# Autodesk Inventor assembly: formed_machine
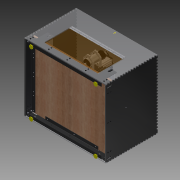
[picture p0: Inventor's stored thumbnail of the model, 180x180]
Saved by Autodesk Inventor 2014 (Build 180170000, 170)
## iProperties
Created: 2013-05-31
Part Number: formed_machine
Document SubType Name: Assembly
Designer: Edward
Mass: 12074.1 g
Surface Area: 21541.8 cm^2
Volume: 5793.23 cm^3
Density: 2.08417 g/cm^3
Author: Edward
## Documents named in this file (21)
- C:\Users\Edward\Desktop\Shapeoko_2.0_collection\Shapeoko_formed\Workgroups\Workgroup\shapeoko_v2_0.iam
- C:\Users\Edward\Desktop\Shapeoko_2.0_collection\Shapeoko_formed\Workgroups\Workgroup\formed_front_back.ipt
- C:\Users\Edward\Desktop\Shapeoko_2.0_collection\Shapeoko_formed\Workgroups\Workgroup\S2_MS500.ipt
- C:\Users\Edward\Desktop\Shapeoko_2.0_collection\Shapeoko_formed\Workgroups\Workgroup\plate_assembly_stacked.iam
- C:\Users\Edward\Desktop\Shapeoko_2.0_collection\Shapeoko_formed\Workgroups\Workgroup\formed_right_left.ipt
- C:\Users\Edward\Desktop\Shapeoko_2.0_collection\Shapeoko_formed\Workgroups\Workgroup\sectional_wasteboard.ipt
- C:\Users\Edward\Desktop\Shapeoko_2.0_collection\Shapeoko_formed\Workgroups\Workgroup\23015T82_leveling_feet.ipt
- C:\Users\Edward\Desktop\Shapeoko_2.0_collection\Shapeoko_formed\Workgroups\Workgroup\z-axis_assembly.iam
- C:\Users\Edward\Desktop\Shapeoko_2.0_collection\Shapeoko_formed\Workgroups\Workgroup\SM-H03.ipt
- C:\Users\Edward\Desktop\Shapeoko_2.0_collection\Shapeoko_formed\Workgroups\Workgroup\SM-H04.ipt
- C:\Users\Edward\Desktop\Shapeoko_2.0_collection\Shapeoko_formed\Workgroups\Workgroup\91239A228.ipt
- C:\Users\Edward\Desktop\Shapeoko_2.0_collection\Shapeoko_formed\Workgroups\Workgroup\belt_clip_assembly.iam
- C:\Users\Edward\Desktop\Shapeoko_2.0_collection\Shapeoko_formed\Workgroups\Workgroup\97349A200.ipt
- C:\Users\Edward\Desktop\Shapeoko_2.0_collection\Shapeoko_formed\Workgroups\Workgroup\GT2_XY_belting.ipt
- C:\Users\Edward\Desktop\Shapeoko_2.0_collection\Shapeoko_formed\Workgroups\Workgroup\fr.ipt
- C:\Users\Edward\Desktop\Shapeoko_2.0_collection\Shapeoko_formed\Workgroups\Workgroup\hblsd_assembly.iam
- C:\Users\Edward\Desktop\Shapeoko_2.0_collection\Shapeoko_formed\Workgroups\Workgroup\case_right.ipt
- C:\Users\Edward\Desktop\Shapeoko_2.0_collection\Shapeoko_formed\Workgroups\Workgroup\case_front.ipt
- C:\Users\Edward\Desktop\Shapeoko_2.0_collection\Shapeoko_formed\Workgroups\Workgroup\case_rear.ipt
- C:\Users\Edward\Desktop\Shapeoko_2.0_collection\Shapeoko_formed\Workgroups\Workgroup\Imported Components\1569A107\1569A107.ipt
- C:\Users\Edward\Desktop\Shapeoko_2.0_collection\Shapeoko_formed\Workgroups\Workgroup\case_door.ipt
## Components (159 placed, 20 different names)
1. formed_front_back:1 — Angle:1, Angle:2, Flush:4, Mate:16, Flush:5, Insert:9, Insert:10, Mate:22, Mate:23, Flush:10, Flush:11, Flush:12, Flush:13, Flush:14, Flush:15, Mate:31, Insert:55, Insert:56, Insert:57, Mate:38, Flush:22
2. S2_MS500:1 — Angle:2, Mate:1, Flush:1, Insert:6, Insert:17, Insert:18, Mate:23, Flush:10, Flush:13, Mate:24, Mate:28, Mate:30, Flush:16, Mate:43, Flush:26
3. plate_assembly_stacked:1 [sub-assembly] — Mate:1, Flush:1, Insert:4, Angle:3, Mate:36
4. S2_MS500:2 — Angle:1, Mate:2, Flush:2, Insert:5, Insert:23, Insert:24, Mate:22, Flush:11, Flush:12, Mate:25, Mate:27, Mate:41
5. plate_assembly_stacked:2 [sub-assembly] — Mate:2, Flush:2, Insert:3, Mate:34
6. S2_MS500:3 — Insert:3, Insert:4, Mate:20, Flush:7, Angle:3, Insert:37, Insert:38, Insert:40, Insert:42, Mate:21, Mate:26, Mate:29, Mate:33, Mate:35, Flush:18, Flush:19, Mate:42, Flush:25
7. formed_front_back:2 — Insert:5, Insert:6, Mate:14, Mate:15, Mate:17, Mate:19, Insert:7, Insert:8, Mate:24, Flush:14, Flush:15, Insert:66, Insert:67, Insert:68, Insert:87, Insert:88
8. formed_right_left:3 — Mate:14, Mate:15, Flush:4, Mate:18, Flush:6, Insert:27, Insert:28, Insert:58, Insert:59, Insert:60, Insert:61, Insert:62, Insert:63, Insert:64, Insert:65, Mate:39, Insert:85, Insert:86
9. formed_right_left:4 — Mate:16, Mate:17, Flush:5, Insert:31, Insert:32, Insert:47, Insert:48, Insert:49, Insert:50, Insert:51, Insert:52, Insert:53, Insert:54, Mate:37, Flush:20, Flush:21
10. 23015T82_leveling_feet:1 — Insert:7
11. 23015T82_leveling_feet:2 — Insert:8
12. 23015T82_leveling_feet:3 — Insert:9
13. 23015T82_leveling_feet:4 — Insert:10
14. z-axis_assembly:1 [sub-assembly] — Mate:20, Flush:7, Flush:8, Flush:9, Mate:32, Flush:17
15. SM-H03:3 — Insert:16, Insert:17
16. SM-H03:4 — Insert:15, Insert:18
17. 91239A228:3 — Insert:15
18. 91239A228:4 — Insert:16
19. 91239A228:5 — Insert:22
20. SM-H03:5 — Insert:22, Insert:23
21. 91239A228:6 — Insert:21
22. SM-H03:6 — Insert:21, Insert:24
23. 91239A228:11 — Insert:35
24. SM-H03:11 — Insert:35, Insert:37
25. 91239A228:12 — Insert:36
26. SM-H03:12 — Insert:36, Insert:38
27. 91239A228:13 — Insert:41
28. SM-H03:13 — Insert:41, Insert:42
29. 91239A228:14 — Insert:39
30. SM-H03:14 — Insert:39, Insert:40
31. plate_assembly_stacked:3 [sub-assembly] — Mate:21, Flush:8, Flush:9
32. belt_clip_assembly:1 [sub-assembly] — Mate:25
33. belt_clip_assembly:2 [sub-assembly] — Mate:26
34. belt_clip_assembly:3 [sub-assembly] — Mate:27
35. belt_clip_assembly:4 [sub-assembly] — Mate:28
36. belt_clip_assembly:5 [sub-assembly] — Mate:29
37. belt_clip_assembly:6 [sub-assembly] — Mate:30, Mate:31, Flush:16
38. 97349A200:1 — Insert:47
39. 97349A200:2 — Insert:49
40. 97349A200:3 — Insert:48
41. 97349A200:4 — Insert:50
42. 97349A200:5 — Insert:51
43. 97349A200:6 — Insert:52
44. 97349A200:7 — Insert:53
45. 97349A200:8 — Insert:54
46. 97349A200:9 — Insert:57
47. 97349A200:10 — Insert:56
48. 97349A200:11 — Insert:55
49. 97349A200:12 — Insert:58
50. 97349A200:13 — Insert:60
51. 97349A200:14 — Insert:59
52. 97349A200:15 — Insert:62
53. 97349A200:16 — Insert:61
54. 97349A200:17 — Insert:64
55. 97349A200:18 — Insert:63
56. 97349A200:19 — Insert:65
57. 97349A200:20 — Insert:66
58. 97349A200:21 — Insert:67
59. 97349A200:22 — Insert:68
60. GT2_XY_belting:1 — Mate:41
61. GT2_XY_belting:2 — Mate:42, Flush:25
62. GT2_XY_belting:3 — Mate:43, Flush:26
63. fr:1 — Mate:32, Flush:17
64. hblsd_assembly:1 [sub-assembly] — Mate:35, Mate:36, Flush:18, Insert:75, Insert:76, Insert:79, Insert:80
65. hblsd_assembly:2 [sub-assembly] — Mate:33, Mate:34, Flush:19, Insert:70, Insert:72, Insert:83, Insert:84
66. 91239A228:19 — Insert:69
67. SM-H03:25 — Insert:69, Insert:70
68. 91239A228:20 — Insert:71
69. SM-H03:26 — Insert:71, Insert:72
70. 91239A228:21 — Insert:73
71. SM-H03:27 — Insert:73, Insert:76
72. 91239A228:22 — Insert:74
73. SM-H03:28 — Insert:74, Insert:75
74. SM-H03:29 — Insert:77, Insert:80
75. SM-H04:9 — Insert:77
76. SM-H03:30 — Insert:78, Insert:79
77. SM-H04:10 — Insert:78
78. SM-H03:31 — Insert:81, Insert:84
79. SM-H04:11 — Insert:81
80. SM-H03:32 — Insert:82, Insert:83
81. SM-H04:12 — Insert:82
82. case_right:1 — Flush:21, Insert:91
83. case_right:2 — Mate:39, Insert:85, Insert:86, Flush:23, Insert:112
84. case_front:1 — Flush:22, Mate:40, Flush:24, Insert:92, Insert:93, Insert:94, Insert:95, Insert:96, Insert:97, Insert:98, Insert:99, Insert:100, Insert:101
85. case_rear:1 — Insert:87, Insert:88, Insert:102, Insert:103, Insert:104, Insert:105, Insert:106, Insert:107, Insert:108, Insert:109, Insert:110, Insert:111
86. 1569A107:1 — Mate:40, Flush:23, Flush:24, Insert:89, Insert:90
87. case_door:1 — Insert:89, Insert:90
88. 91239A228:30 — Insert:92
89. 91239A228:31 — Insert:93
90. 91239A228:32 — Insert:94
91. 91239A228:33 — Insert:95
92. 91239A228:34 — Insert:96
93. 91239A228:35 — Insert:97
94. 91239A228:36 — Insert:98
95. 91239A228:37 — Insert:99
96. 91239A228:38 — Insert:100
97. 91239A228:39 — Insert:101
98. 91239A228:40 — Insert:103
99. 91239A228:41 — Insert:102
100. 91239A228:42 — Insert:110
101. 91239A228:43 — Insert:111
102. 91239A228:44 — Insert:108
103. 91239A228:45 — Insert:109
104. 91239A228:46 — Insert:106
105. 91239A228:47 — Insert:107
106. 91239A228:48 — Insert:104
107. 91239A228:49 — Insert:105
108. sectional_wasteboard:2 — Mate:18, Flush:6, Mate:19
109. sectional_wasteboard:3
110. sectional_wasteboard:4
111. sectional_wasteboard:5
112. SM-H04:1 — Insert:11
113. SM-H03:1 — Insert:11, Insert:33
114. SM-H04:2 — Insert:12
115. SM-H03:2 — Insert:12, Insert:34
116. SM-H03:9 — Insert:30, Insert:31
117. 91239A228:9 — Insert:30, Insert:33
118. SM-H03:10 — Insert:29, Insert:32
119. 91239A228:10 — Insert:29, Insert:34
120. SM-H04:3
121. SM-H03:15
122. SM-H04:4
123. SM-H03:16
124. SM-H03:17
125. 91239A228:15
126. SM-H03:18
127. 91239A228:16
128. 91239A228:7 — Insert:26, Insert:44
129. SM-H03:7 — Insert:26, Insert:27
130. SM-H03:8 — Insert:25, Insert:28
131. 91239A228:8 — Insert:25, Insert:46
132. SM-H04:6 — Insert:43
133. SM-H03:20 — Insert:43, Insert:44
134. SM-H03:19 — Insert:45, Insert:46
135. SM-H04:5 — Insert:45
136. 91239A228:17
137. SM-H03:21
138. SM-H03:22
139. 91239A228:18
140. SM-H04:7
141. SM-H03:23
142. SM-H03:24
143. SM-H04:8
144. sectional_wasteboard:6 — Mate:37, Flush:20, Mate:38
145. sectional_wasteboard:7
146. sectional_wasteboard:8
147. sectional_wasteboard:9
148. 91239A228:24 — Insert:91
149. 91239A228:25
150. 91239A228:26
151. 91239A228:27
152. 91239A228:28
153. 91239A228:29
154. 91239A228:51 — Insert:112
155. 91239A228:52
156. 91239A228:53
157. 91239A228:54
158. 91239A228:55
159. 91239A228:56
## Component patterns: (4 elements, first: sectional_wasteboard:2), (2 elements, first: SM-H04:1 + SM-H03:1 + SM-H04:2 + SM-H03:2 + SM-H03:9 + 91239A228:9 + SM-H03:10 + 91239A228:10), (2 elements, first: 91239A228:7 + SM-H03:7 + SM-H03:8 + 91239A228:8 + SM-H04:6 + SM-H03:20 + SM-H03:19 + SM-H04:5), (4 elements, first: sectional_wasteboard:6), (6 elements, first: 91239A228:24), (6 elements, first: 91239A228:51)
## Relationships (166: Insert 106, Mate 32, Flush 25, Angle 3)
- Angle:1 (0 deg): formed_front_back:1 ↔ S2_MS500:2
- Angle:2 (0 deg): formed_front_back:1 ↔ S2_MS500:1
- Mate:1 (6.35 mm): S2_MS500:1 ↔ plate_assembly_stacked:1
- Flush:1 (-25 mm): S2_MS500:1 ↔ plate_assembly_stacked:1
- Mate:2 (6.35 mm): S2_MS500:2 ↔ plate_assembly_stacked:2
- Flush:2 (-25 mm): S2_MS500:2 ↔ plate_assembly_stacked:2
- Insert:3: plate_assembly_stacked:2 ↔ S2_MS500:3
- Insert:4: plate_assembly_stacked:1 ↔ S2_MS500:3
- Insert:5: S2_MS500:2 ↔ formed_front_back:2
- Insert:6: S2_MS500:1 ↔ formed_front_back:2
- Mate:14: formed_front_back:2 ↔ formed_right_left:3
- Mate:15 (5 mm): formed_front_back:2 ↔ formed_right_left:3
- Flush:4: formed_front_back:1 ↔ formed_right_left:3
- Mate:16: formed_front_back:1 ↔ formed_right_left:4
- Mate:17 (5 mm): formed_front_back:2 ↔ formed_right_left:4
- Flush:5: formed_front_back:1 ↔ formed_right_left:4
- Mate:18: formed_right_left:3 ↔ sectional_wasteboard:2
- Flush:6 (3 mm): formed_right_left:3 ↔ sectional_wasteboard:2
- Mate:19: formed_front_back:2 ↔ sectional_wasteboard:2
- Insert:7 (6.35 mm): formed_front_back:2 ↔ 23015T82_leveling_feet:1
- Insert:8 (6.35 mm): formed_front_back:2 ↔ 23015T82_leveling_feet:2
- Insert:9 (6.35 mm): formed_front_back:1 ↔ 23015T82_leveling_feet:3
- Insert:10 (6.35 mm): formed_front_back:1 ↔ 23015T82_leveling_feet:4
- Mate:20 (6.35 mm): S2_MS500:3 ↔ z-axis_assembly:1
- Flush:7 (-25 mm): S2_MS500:3 ↔ z-axis_assembly:1
- Angle:3 (0 deg): plate_assembly_stacked:1 ↔ S2_MS500:3
- Insert:11: SM-H04:1 ↔ SM-H03:1
- Insert:12: SM-H04:2 ↔ SM-H03:2
- Insert:15: SM-H03:4 ↔ 91239A228:3
- Insert:16: SM-H03:3 ↔ 91239A228:4
- Insert:17 (3 mm): S2_MS500:1 ↔ SM-H03:3
- Insert:18 (3 mm): S2_MS500:1 ↔ SM-H03:4
- Insert:21: 91239A228:6 ↔ SM-H03:6
- Insert:22: 91239A228:5 ↔ SM-H03:5
- Insert:23 (3 mm): S2_MS500:2 ↔ SM-H03:5
- Insert:24 (3 mm): S2_MS500:2 ↔ SM-H03:6
- Insert:25: SM-H03:8 ↔ 91239A228:8
- Insert:26: 91239A228:7 ↔ SM-H03:7
- Insert:27: formed_right_left:3 ↔ SM-H03:7
- Insert:28: formed_right_left:3 ↔ SM-H03:8
- Insert:29: SM-H03:10 ↔ 91239A228:10
- Insert:30: SM-H03:9 ↔ 91239A228:9
- Insert:31: formed_right_left:4 ↔ SM-H03:9
- Insert:32: formed_right_left:4 ↔ SM-H03:10
- Insert:33 (-5 mm): SM-H03:1 ↔ 91239A228:9
- Insert:34 (-5 mm): SM-H03:2 ↔ 91239A228:10
- Insert:35: 91239A228:11 ↔ SM-H03:11
- Insert:36: 91239A228:12 ↔ SM-H03:12
- Insert:37 (4 mm): S2_MS500:3 ↔ SM-H03:11
- Insert:38 (4 mm): S2_MS500:3 ↔ SM-H03:12
- Insert:39: 91239A228:14 ↔ SM-H03:14
- Insert:40 (4 mm): S2_MS500:3 ↔ SM-H03:14
- Insert:41: 91239A228:13 ↔ SM-H03:13
- Insert:42 (4 mm): S2_MS500:3 ↔ SM-H03:13
- Insert:43: SM-H04:6 ↔ SM-H03:20
- Insert:44 (-5 mm): 91239A228:7 ↔ SM-H03:20
- Insert:45: SM-H03:19 ↔ SM-H04:5
- Insert:46 (-5 mm): 91239A228:8 ↔ SM-H03:19
- Mate:21 (6.35 mm): S2_MS500:3 ↔ plate_assembly_stacked:3
- Flush:8: z-axis_assembly:1 ↔ plate_assembly_stacked:3
- Flush:9: z-axis_assembly:1 ↔ plate_assembly_stacked:3
- Mate:22: formed_front_back:1 ↔ S2_MS500:2
- Mate:23: formed_front_back:1 ↔ S2_MS500:1
- Flush:10: formed_front_back:1 ↔ S2_MS500:1
- Flush:11: formed_front_back:1 ↔ S2_MS500:2
- Flush:12 (20 mm): formed_front_back:1 ↔ S2_MS500:2
- Flush:13 (20 mm): formed_front_back:1 ↔ S2_MS500:1
- Mate:24: S2_MS500:1 ↔ formed_front_back:2
- Flush:14: formed_front_back:1 ↔ formed_front_back:2
- Flush:15: formed_front_back:1 ↔ formed_front_back:2
- Mate:25: S2_MS500:2 ↔ belt_clip_assembly:1
- Mate:26: S2_MS500:3 ↔ belt_clip_assembly:2
- Mate:27: S2_MS500:2 ↔ belt_clip_assembly:3
- Mate:28: S2_MS500:1 ↔ belt_clip_assembly:4
- Mate:29: S2_MS500:3 ↔ belt_clip_assembly:5
- Mate:30: S2_MS500:1 ↔ belt_clip_assembly:6
- Mate:31: formed_front_back:1 ↔ belt_clip_assembly:6
- Flush:16 (2 mm): S2_MS500:1 ↔ belt_clip_assembly:6
- Insert:47: formed_right_left:4 ↔ 97349A200:1
- Insert:48: formed_right_left:4 ↔ 97349A200:3
- Insert:49: formed_right_left:4 ↔ 97349A200:2
- Insert:50: formed_right_left:4 ↔ 97349A200:4
- Insert:51: formed_right_left:4 ↔ 97349A200:5
- Insert:52: formed_right_left:4 ↔ 97349A200:6
- Insert:53: formed_right_left:4 ↔ 97349A200:7
- Insert:54: formed_right_left:4 ↔ 97349A200:8
- Insert:55: formed_front_back:1 ↔ 97349A200:11
- Insert:56: formed_front_back:1 ↔ 97349A200:10
- Insert:57: formed_front_back:1 ↔ 97349A200:9
- Insert:58: formed_right_left:3 ↔ 97349A200:12
- Insert:59: formed_right_left:3 ↔ 97349A200:14
- Insert:60: formed_right_left:3 ↔ 97349A200:13
- Insert:61: formed_right_left:3 ↔ 97349A200:16
- Insert:62: formed_right_left:3 ↔ 97349A200:15
- Insert:63: formed_right_left:3 ↔ 97349A200:18
- Insert:64: formed_right_left:3 ↔ 97349A200:17
- Insert:65: formed_right_left:3 ↔ 97349A200:19
- Insert:66: formed_front_back:2 ↔ 97349A200:20
- Insert:67: formed_front_back:2 ↔ 97349A200:21
- Insert:68: formed_front_back:2 ↔ 97349A200:22
- Mate:32: z-axis_assembly:1 ↔ fr:1
- Flush:17 (-45 mm): z-axis_assembly:1 ↔ fr:1
- Mate:33: S2_MS500:3 ↔ hblsd_assembly:2
- Mate:34: plate_assembly_stacked:2 ↔ hblsd_assembly:2
- Mate:35: S2_MS500:3 ↔ hblsd_assembly:1
- Mate:36: plate_assembly_stacked:1 ↔ hblsd_assembly:1
- Flush:18 (3 mm): S2_MS500:3 ↔ hblsd_assembly:1
- Flush:19 (3 mm): S2_MS500:3 ↔ hblsd_assembly:2
- Insert:69: 91239A228:19 ↔ SM-H03:25
- Insert:70 (4 mm): hblsd_assembly:2 ↔ SM-H03:25
- Insert:71: 91239A228:20 ↔ SM-H03:26
- Insert:72 (4 mm): hblsd_assembly:2 ↔ SM-H03:26
- Insert:73: 91239A228:21 ↔ SM-H03:27
- Insert:74: 91239A228:22 ↔ SM-H03:28
- Insert:75 (4 mm): hblsd_assembly:1 ↔ SM-H03:28
- Insert:76 (4 mm): hblsd_assembly:1 ↔ SM-H03:27
- Insert:77: SM-H03:29 ↔ SM-H04:9
- Insert:78: SM-H03:30 ↔ SM-H04:10
- Insert:79: hblsd_assembly:1 ↔ SM-H03:30
- Insert:80: hblsd_assembly:1 ↔ SM-H03:29
- Insert:81: SM-H03:31 ↔ SM-H04:11
- Insert:82: SM-H03:32 ↔ SM-H04:12
- Insert:83: hblsd_assembly:2 ↔ SM-H03:32
- Insert:84: hblsd_assembly:2 ↔ SM-H03:31
- Mate:37: formed_right_left:4 ↔ sectional_wasteboard:6
- Flush:20: formed_right_left:4 ↔ sectional_wasteboard:6
- Mate:38: formed_front_back:1 ↔ sectional_wasteboard:6
- Flush:21: formed_right_left:4 ↔ case_right:1
- Mate:39: formed_right_left:3 ↔ case_right:2
- Insert:85: formed_right_left:3 ↔ case_right:2
- Insert:86: formed_right_left:3 ↔ case_right:2
- Flush:22: formed_front_back:1 ↔ case_front:1
- Insert:87: formed_front_back:2 ↔ case_rear:1
- Insert:88: formed_front_back:2 ↔ case_rear:1
- Mate:40: case_front:1 ↔ 1569A107:1
- Flush:23 (106.15 mm): case_right:2 ↔ 1569A107:1
- Flush:24 (-12.7 mm): case_front:1 ↔ 1569A107:1
- Insert:89: 1569A107:1 ↔ case_door:1
- Insert:90: 1569A107:1 ↔ case_door:1
- Insert:91: case_right:1 ↔ 91239A228:24
- Insert:92: case_front:1 ↔ 91239A228:30
- Insert:93: case_front:1 ↔ 91239A228:31
- Insert:94: case_front:1 ↔ 91239A228:32
- Insert:95: case_front:1 ↔ 91239A228:33
- Insert:96: case_front:1 ↔ 91239A228:34
- Insert:97: case_front:1 ↔ 91239A228:35
- Insert:98: case_front:1 ↔ 91239A228:36
- Insert:99: case_front:1 ↔ 91239A228:37
- Insert:100: case_front:1 ↔ 91239A228:38
- Insert:101: case_front:1 ↔ 91239A228:39
- Insert:102: case_rear:1 ↔ 91239A228:41
- Insert:103: case_rear:1 ↔ 91239A228:40
- Insert:104: case_rear:1 ↔ 91239A228:48
- Insert:105: case_rear:1 ↔ 91239A228:49
- Insert:106: case_rear:1 ↔ 91239A228:46
- Insert:107: case_rear:1 ↔ 91239A228:47
- Insert:108: case_rear:1 ↔ 91239A228:44
- Insert:109: case_rear:1 ↔ 91239A228:45
- Insert:110: case_rear:1 ↔ 91239A228:42
- Insert:111: case_rear:1 ↔ 91239A228:43
- Insert:112: case_right:2 ↔ 91239A228:51
- Mate:41: S2_MS500:2 ↔ GT2_XY_belting:1
- Mate:42: S2_MS500:3 ↔ GT2_XY_belting:2
- Flush:25 (6 mm): S2_MS500:3 ↔ GT2_XY_belting:2
- Mate:43: S2_MS500:1 ↔ GT2_XY_belting:3
- Flush:26 (7 mm): S2_MS500:1 ↔ GT2_XY_belting:3
